# Autodesk Inventor assembly: RoboticArm
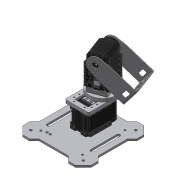
[picture p0: Inventor's stored thumbnail of the model, 180x180]
Saved by Autodesk Inventor 2018 (Build 220112000, 112)
## iProperties
Created: 2021-01-30
Part Number: RoboticArm
Material: Ogólny
Document SubType Name: Assembly
Designer: Marzena
Mass: 128.669 g
Surface Area: 625.59 cm^2
Volume: 128.669 cm^3
Density: 1 g/cm^3
Author: Marzena
## Documents named in this file (4)
- C:\Users\Marzena\Desktop\ControlArduinoByInventorModel\InventorRoboticArmModels\RoboticArm.iam
- C:\Users\Marzena\Desktop\ControlArduinoByInventorModel\InventorRoboticArmModels\Part1.ipt
- C:\Users\Marzena\Desktop\ControlArduinoByInventorModel\InventorRoboticArmModels\Part2.ipt
- C:\Users\Marzena\Desktop\ControlArduinoByInventorModel\InventorRoboticArmModels\Part3.ipt
## Components (3 placed, 3 different names)
1. Part1:1 — Wstaw:1, Walcowe:1
2. Part2:1 — Wstaw:1, Walcowe:1, Obrotowe:1
3. Part3:1 — Obrotowe:1
## Relationships (3: Insert 1, CylindricalJoint 1, RevoluteJoint 1)
- Wstaw:1 [Insert]: Part1:1 ↔ Part2:1
- Walcowe:1 [CylindricalJoint]: Part1:1 ↔ Part2:1
- Obrotowe:1 [RevoluteJoint]: Part2:1 ↔ Part3:1
